# Autodesk Inventor assembly: autoarm assembly
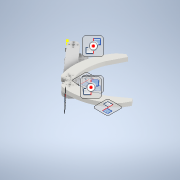
[picture p0: Inventor's stored thumbnail of the model, 180x180]
Saved by Autodesk Inventor 2020 (Build 240168000, 168)
## iProperties
Created: 2020-01-21
Part Number: autoarm assembly
Document SubType Name: Assembly
Designer: piolo.pulanco
Author: piolo.pulanco
## Documents named in this file (7)
- C:\Users\tdmp4\OneDrive\Documents\GitHub\CAD-2020\autoarm assembly.iam
- C:\Users\tdmp4\OneDrive\Documents\GitHub\CAD-2020\Autoarm parts\Spur Gear15.ipt
- C:\Users\tdmp4\OneDrive\Documents\GitHub\CAD-2020\Autoarm parts\Claw arm.ipt
- C:\Users\tdmp4\OneDrive\Documents\GitHub\CAD-2020\Autoarm parts\REV-41-1097.ipt
- C:\Users\tdmp4\OneDrive\Documents\GitHub\CAD-2020\Autoarm parts\REV-41-1363.ipt
- C:\Users\tdmp4\OneDrive\Documents\GitHub\CAD-2020\ServoCity\Servo Block.iam
- C:\Users\tdmp4\OneDrive\Documents\GitHub\CAD-2020\Autoarm parts\Spur Gear15_MIR.ipt
## Components (6 placed, 6 different names)
1. Spur Gear1:1 — Mate:22, Mate:24
2. Claw arm:1 — Mate:17, Mate:18, Mate:26, Mate:27, Mate:28, Mate:29
3. REV-41-1097:2 — Mate:17, Mate:18, Mate:20, Mate:21
4. Spur Gear15_MIR:1 — Mate:26, Mate:27
5. REV-41-1363:1 — Mate:20, Mate:21, Mate:22, Mate:24
6. Servo Block:1 [sub-assembly] — Mate:28, Mate:29
## Relationships (10: Mate 10)
- Mate:17: Claw arm:1 ↔ REV-41-1097:2
- Mate:18: Claw arm:1 ↔ REV-41-1097:2
- Mate:20: REV-41-1097:2 ↔ REV-41-1363:1
- Mate:21: REV-41-1097:2 ↔ REV-41-1363:1
- Mate:22: Spur Gear1:1 ↔ REV-41-1363:1
- Mate:24: Spur Gear1:1 ↔ REV-41-1363:1
- Mate:26: Claw arm:1 ↔ Spur Gear15_MIR:1
- Mate:27 (5.08 mm): Claw arm:1 ↔ Spur Gear15_MIR:1
- Mate:28: Claw arm:1 ↔ Servo Block:1
- Mate:29: Claw arm:1 ↔ Servo Block:1
